# Autodesk Inventor assembly: AM14U3 Long Frame Half
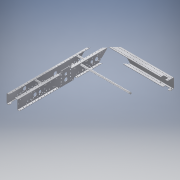
[picture p0: Inventor's stored thumbnail of the model, 180x180]
Saved by Autodesk Inventor 2016 (Build 200138000, 138)
## iProperties
Created: 2016-01-13
Part Number: AM14U3 Long Frame Half
Document SubType Name: Assembly
Designer: Douglas
Author: Douglas
Revision Number: ANY
## Documents named in this file (9)
- D:\SkyDrive\GitHub\2016-Robot-CAD\Inventor\Chassis\AM14U3 Long Frame Half.iam
- D:\SkyDrive\GitHub\2016-Robot-CAD\Inventor\Chassis\Churro 3375.ipt
- D:\SkyDrive\GitHub\2016-Robot-CAD\Inventor\Chassis\FHTS 0.25-20-0.75_FHTS 0.25-20-G-0.75-C.ipt
- D:\SkyDrive\GitHub\2016-Robot-CAD\Inventor\Chassis\Churro 16250.ipt
- D:\SkyDrive\GitHub\2016-Robot-CAD\Inventor\Chassis\10-32x0500_shcs_HX-SHCS 0.19-32x1.375x1-C.ipt
- D:\SkyDrive\GitHub\2016-Robot-CAD\Inventor\Chassis\10-32 Nylock Nut.ipt
- D:\SkyDrive\GitHub\2016-Robot-CAD\Inventor\Chassis\AM14U3 End Sheet Long.ipt
- D:\SkyDrive\GitHub\2016-Robot-CAD\Inventor\Chassis\AM14U3 Inside Sheet Rev2.ipt
- D:\SkyDrive\GitHub\2016-Robot-CAD\Inventor\Chassis\AM14U3 Outside Sheet Rev1_DefaultSM-FLAT-PATTERN.ipt
## Components (26 placed, 26 different names)
1. Churro 3375_80 — Mate:1, Mate:2, Mate:3, Mate:5
2. Churro 3375_81 — Mate:58, Mate:59, Mate:60, Mate:62
3. Churro 3375_82 — Mate:7, Mate:8, Mate:9, Mate:10
4. Churro 3375_83 — Mate:52, Mate:53, Mate:54, Mate:55
5. FHTS 0.25-20-0.75_FHTS 0.25-20-G-0.75-C_84 — Mate:60, Mate:61
6. FHTS 0.25-20-0.75_FHTS 0.25-20-G-0.75-C_85 — Mate:3, Mate:4
7. FHTS 0.25-20-0.75_FHTS 0.25-20-G-0.75-C_86 — Mate:9, Mate:12
8. FHTS 0.25-20-0.75_FHTS 0.25-20-G-0.75-C_87 — Mate:55, Mate:56
9. FHTS 0.25-20-0.75_FHTS 0.25-20-G-0.75-C_88 — Mate:62, Mate:63
10. FHTS 0.25-20-0.75_FHTS 0.25-20-G-0.75-C_89 — Mate:5, Mate:6
11. FHTS 0.25-20-0.75_FHTS 0.25-20-G-0.75-C_90 — Mate:54, Mate:57
12. FHTS 0.25-20-0.75_FHTS 0.25-20-G-0.75-C_91 — Mate:10, Mate:11
13. FHTS 0.25-20-0.75_FHTS 0.25-20-G-0.75-C_92
14. FHTS 0.25-20-0.75_FHTS 0.25-20-G-0.75-C_93
15. Churro 16250_94
16. 10-32x0500_shcs_HX-SHCS 0.19-32x1.375x1-C_99 — Mate:84, Mate:85, Mate:88
17. 10-32x0500_shcs_HX-SHCS 0.19-32x1.375x1-C_100 — Mate:83, Mate:86, Mate:87
18. 10-32x0500_shcs_HX-SHCS 0.19-32x1.375x1-C_105
19. 10-32x0500_shcs_HX-SHCS 0.19-32x1.375x1-C_106
20. 10-32 Nylock Nut_111
21. 10-32 Nylock Nut_112
22. 10-32 Nylock Nut_117 — Mate:88, Mate:90
23. 10-32 Nylock Nut_118 — Mate:87, Mate:89
24. AM14U3 End Sheet Long_135 — Mate:64, Mate:65, Mate:66, Mate:83, Mate:89, Mate:90
25. AM14U3 Inside Sheet Rev2_136 — Mate:1, Mate:2, Mate:4, Mate:7, Mate:8, Mate:12, Mate:52, Mate:56, Mate:58, Mate:61, Mate:64, Mate:84, Mate:85
26. AM14U3 Outside Sheet Rev1_DefaultSM-FLAT-PATTERN_137 — Mate:6, Mate:11, Mate:53, Mate:57, Mate:59, Mate:63, Mate:65, Mate:66, Mate:86
## Relationships (35: Mate 35)
- Mate:1: Churro 3375_80 ↔ AM14U3 Inside Sheet Rev2_136
- Mate:2: Churro 3375_80 ↔ AM14U3 Inside Sheet Rev2_136
- Mate:3: Churro 3375_80 ↔ FHTS 0.25-20-0.75_FHTS 0.25-20-G-0.75-C_85
- Mate:4: FHTS 0.25-20-0.75_FHTS 0.25-20-G-0.75-C_85 ↔ AM14U3 Inside Sheet Rev2_136
- Mate:5: Churro 3375_80 ↔ FHTS 0.25-20-0.75_FHTS 0.25-20-G-0.75-C_89
- Mate:6: FHTS 0.25-20-0.75_FHTS 0.25-20-G-0.75-C_89 ↔ AM14U3 Outside Sheet Rev1_DefaultSM-FLAT-PATTERN_137
- Mate:7: Churro 3375_82 ↔ AM14U3 Inside Sheet Rev2_136
- Mate:8: Churro 3375_82 ↔ AM14U3 Inside Sheet Rev2_136
- Mate:9: Churro 3375_82 ↔ FHTS 0.25-20-0.75_FHTS 0.25-20-G-0.75-C_86
- Mate:10: Churro 3375_82 ↔ FHTS 0.25-20-0.75_FHTS 0.25-20-G-0.75-C_91
- Mate:11: FHTS 0.25-20-0.75_FHTS 0.25-20-G-0.75-C_91 ↔ AM14U3 Outside Sheet Rev1_DefaultSM-FLAT-PATTERN_137
- Mate:12: FHTS 0.25-20-0.75_FHTS 0.25-20-G-0.75-C_86 ↔ AM14U3 Inside Sheet Rev2_136
- Mate:52: Churro 3375_83 ↔ AM14U3 Inside Sheet Rev2_136
- Mate:53: Churro 3375_83 ↔ AM14U3 Outside Sheet Rev1_DefaultSM-FLAT-PATTERN_137
- Mate:54: Churro 3375_83 ↔ FHTS 0.25-20-0.75_FHTS 0.25-20-G-0.75-C_90
- Mate:55: Churro 3375_83 ↔ FHTS 0.25-20-0.75_FHTS 0.25-20-G-0.75-C_87
- Mate:56: FHTS 0.25-20-0.75_FHTS 0.25-20-G-0.75-C_87 ↔ AM14U3 Inside Sheet Rev2_136
- Mate:57: FHTS 0.25-20-0.75_FHTS 0.25-20-G-0.75-C_90 ↔ AM14U3 Outside Sheet Rev1_DefaultSM-FLAT-PATTERN_137
- Mate:58: Churro 3375_81 ↔ AM14U3 Inside Sheet Rev2_136
- Mate:59: Churro 3375_81 ↔ AM14U3 Outside Sheet Rev1_DefaultSM-FLAT-PATTERN_137
- Mate:60: Churro 3375_81 ↔ FHTS 0.25-20-0.75_FHTS 0.25-20-G-0.75-C_84
- Mate:61: FHTS 0.25-20-0.75_FHTS 0.25-20-G-0.75-C_84 ↔ AM14U3 Inside Sheet Rev2_136
- Mate:62: Churro 3375_81 ↔ FHTS 0.25-20-0.75_FHTS 0.25-20-G-0.75-C_88
- Mate:63: FHTS 0.25-20-0.75_FHTS 0.25-20-G-0.75-C_88 ↔ AM14U3 Outside Sheet Rev1_DefaultSM-FLAT-PATTERN_137
- Mate:64: AM14U3 End Sheet Long_135 ↔ AM14U3 Inside Sheet Rev2_136
- Mate:65: AM14U3 End Sheet Long_135 ↔ AM14U3 Outside Sheet Rev1_DefaultSM-FLAT-PATTERN_137
- Mate:66: AM14U3 End Sheet Long_135 ↔ AM14U3 Outside Sheet Rev1_DefaultSM-FLAT-PATTERN_137
- Mate:83: 10-32x0500_shcs_HX-SHCS 0.19-32x1.375x1-C_100 ↔ AM14U3 End Sheet Long_135
- Mate:84: 10-32x0500_shcs_HX-SHCS 0.19-32x1.375x1-C_99 ↔ AM14U3 Inside Sheet Rev2_136
- Mate:85: 10-32x0500_shcs_HX-SHCS 0.19-32x1.375x1-C_99 ↔ AM14U3 Inside Sheet Rev2_136
- Mate:86: 10-32x0500_shcs_HX-SHCS 0.19-32x1.375x1-C_100 ↔ AM14U3 Outside Sheet Rev1_DefaultSM-FLAT-PATTERN_137
- Mate:87: 10-32x0500_shcs_HX-SHCS 0.19-32x1.375x1-C_100 ↔ 10-32 Nylock Nut_118
- Mate:88: 10-32x0500_shcs_HX-SHCS 0.19-32x1.375x1-C_99 ↔ 10-32 Nylock Nut_117
- Mate:89: 10-32 Nylock Nut_118 ↔ AM14U3 End Sheet Long_135
- Mate:90: 10-32 Nylock Nut_117 ↔ AM14U3 End Sheet Long_135
